# Autodesk Inventor assembly: PrintheadV1Assembly1
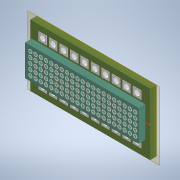
[picture p0: Inventor's stored thumbnail of the model, 180x180]
Saved by Autodesk Inventor 2021 (Build 250183000, 183)
## iProperties
Created: 2022-03-12
Part Number: PrintheadV1Assembly1
Document SubType Name: Assembly
Designer: Unit-005
Author: Unit-005
## Documents named in this file (4)
- C:\Users\Unit-005\Documents\OpenPyrojet\Multipyrojet\PrintheadV1Assembly1.iam
- C:\Users\Unit-005\Documents\Inventor\SiC_Monofilament_MicroheaterPrinthead\2.54mmPitchPerfboardBackplane.ipt
- C:\Users\Unit-005\Documents\Inventor\SiC_Monofilament_MicroheaterPrinthead\1.27mmNozzlePlate v4.ipt
- C:\Users\Unit-005\Documents\OpenPyrojet\Multipyrojet\SiCFilamentRed.ipt
## Components (3 placed, 3 different names)
1. 2.54mmPitchPerfboardBackplane:1 — Mate:1, Mate:2, Tangent:1, Flush:1
2. 1.27mmNozzlePlate v4:1 — Mate:1, Mate:2, Mate:3
3. SiCFilamentRed:1 — Tangent:1, Flush:1, Mate:3
## Relationships (5: Mate 3, Tangent 1, Flush 1)
- Mate:1 (0.135 mm): 2.54mmPitchPerfboardBackplane:1 ↔ 1.27mmNozzlePlate v4:1
- Mate:2: 2.54mmPitchPerfboardBackplane:1 ↔ 1.27mmNozzlePlate v4:1
- Tangent:1: 2.54mmPitchPerfboardBackplane:1 ↔ SiCFilamentRed:1
- Flush:1: 2.54mmPitchPerfboardBackplane:1 ↔ SiCFilamentRed:1
- Mate:3: 1.27mmNozzlePlate v4:1 ↔ SiCFilamentRed:1
